# Autodesk Inventor assembly: Engine Assembly
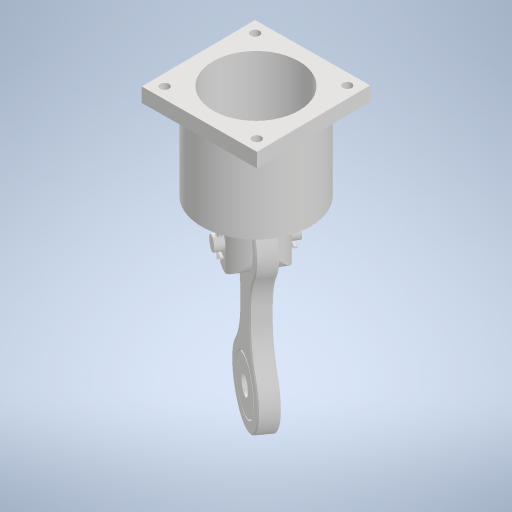
[picture p0: Inventor's stored thumbnail of the model, 512x512]
Saved by Autodesk Inventor 2023 (Build 270158000, 158)
## iProperties
Created: 2022-12-22
Part Number: Engine Assembly
Document SubType Name: Assembly
Designer: tgr41
Author: tgr41
## Documents named in this file (4)
- C:\Users\tgr41\OneDrive\Documents\Repositories\Steam-Engine\2 Inch V3\Engine Assembly.iam
- C:\Users\tgr41\OneDrive\Documents\Repositories\Steam-Engine\2 Inch V3\Piston Subassembly.iam
- C:\Users\tgr41\OneDrive\Documents\Repositories\Steam-Engine\2 Inch V3\Connecting Rod.iam
- C:\Users\tgr41\OneDrive\Documents\Repositories\Steam-Engine\2 Inch V3\Cylinders.ipt
## Components (3 placed, 3 different names)
1. Piston Subassembly:1 [sub-assembly] — Mate:1, Mate:2, Mate:3, Flush:1
2. Connecting Rod:1 [sub-assembly] — Mate:1, Mate:2
3. Cylinders:1 — Mate:3, Flush:1
## Relationships (4: Mate 3, Flush 1)
- Mate:1: Piston Subassembly:1 ↔ Connecting Rod:1
- Mate:2: Piston Subassembly:1 ↔ Connecting Rod:1
- Mate:3: Piston Subassembly:1 ↔ Cylinders:1
- Flush:1: Piston Subassembly:1 ↔ Cylinders:1
